# Autodesk Inventor assembly: 000.700 - Захват
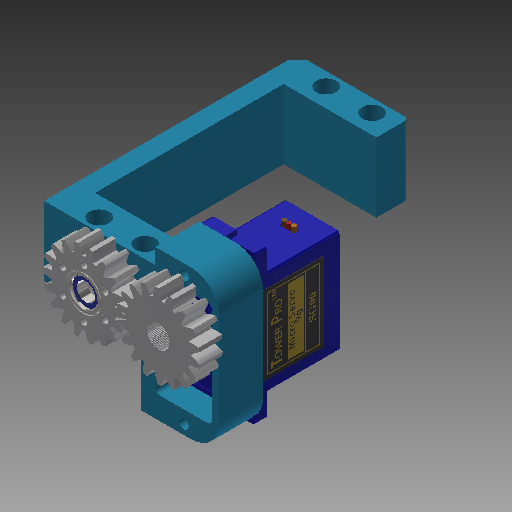
[picture p0: Inventor's stored thumbnail of the model, 512x512]
Saved by Autodesk Inventor 2019 (Build 230136000, 136)
## iProperties
Created: 2020-02-29
Part Number: 000.700 - Захват
Material: Типовые
Document SubType Name: Assembly
Designer: Петров Иван
Author: Петров Иван
## Documents named in this file (5)
- E:\IVAN\Ivan_desktop\GitHub\Manipulation_IRS\hardware\5-DOF\000.700 - Крепеж захвата.iam
- E:\IVAN\Ivan_desktop\GitHub\Manipulation_IRS\hardware\5-DOF\000.701 - Опора.ipt
- E:\IVAN\Ivan_desktop\GitHub\Manipulation_IRS\hardware\5-DOF\components\SG90 - Micro Servo 9g - Tower Pro.1.ipt
- E:\IVAN\Ivan_desktop\GitHub\Manipulation_IRS\hardware\5-DOF\000.700 - Захват\Мастер проектирования\Цилиндрическое зубчатое зацепление2.iam
- E:\IVAN\Ivan_desktop\GitHub\Manipulation_IRS\hardware\5-DOF\components\Подшипник 4x8x3.ipt
## Components (4 placed, 4 different names)
1. 000.701 - Опора:1 — Совмещение:2, Совмещение:3, Совмещение:4, Совмещение:6, Совмещение:7, Совмещение:8
2. SG90 - Micro Servo 9g - Tower Pro.1:1 — Совмещение:2, Совмещение:3, Совмещение:4, Совмещение:5
3. Цилиндрическое зубчатое зацепление:1 [sub-assembly] — Совмещение:5, Совмещение:6, Совмещение:7, Совмещение:8, Совмещение:9, Заподлицо:1, Направление навивки:1
4. Подшипник 4x8x3:1 — Совмещение:9, Заподлицо:1, Направление навивки:1
## Relationships (10: Mate 8, Flush 1, RelateRotation 1)
- Совмещение:2 [Mate]: 000.701 - Опора:1 ↔ SG90 - Micro Servo 9g - Tower Pro.1:1
- Совмещение:3 [Mate]: 000.701 - Опора:1 ↔ SG90 - Micro Servo 9g - Tower Pro.1:1
- Совмещение:4 [Mate]: 000.701 - Опора:1 ↔ SG90 - Micro Servo 9g - Tower Pro.1:1
- Совмещение:5 [Mate]: SG90 - Micro Servo 9g - Tower Pro.1:1 ↔ Цилиндрическое зубчатое зацепление:1
- Совмещение:6 [Mate] (0.5 mm): 000.701 - Опора:1 ↔ Цилиндрическое зубчатое зацепление:1
- Совмещение:7 [Mate]: 000.701 - Опора:1 ↔ Цилиндрическое зубчатое зацепление:1
- Совмещение:8 [Mate] (0.5 mm): 000.701 - Опора:1 ↔ Цилиндрическое зубчатое зацепление:1
- Совмещение:9 [Mate]: Цилиндрическое зубчатое зацепление:1 ↔ Подшипник 4x8x3:1
- Заподлицо:1 [Flush]: Цилиндрическое зубчатое зацепление:1 ↔ Подшипник 4x8x3:1
- Направление навивки:1 [RelateRotation] (1 ul): Цилиндрическое зубчатое зацепление:1 ↔ Подшипник 4x8x3:1
